# Autodesk Inventor assembly: Assemblage_chassis_14_11_C
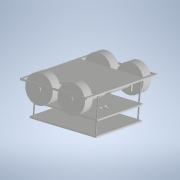
[picture p0: Inventor's stored thumbnail of the model, 180x180]
Saved by Autodesk Inventor 2020.1 (Build 241239000, 239)
## iProperties
Created: 2019-11-14
Part Number: Assemblage_chassis_14_11_C
Document SubType Name: Assembly
Designer: Admin
Author: Admin
## Documents named in this file (7)
- C:\Users\Admin\Desktop\Projet OrangeLab\CAO\Assemblage_chassis_14_11_C.iam
- C:\Users\Admin\Desktop\Projet OrangeLab\CAO\Chassis.ipt
- C:\Users\Admin\Desktop\Projet OrangeLab\CAO\Entretoises 80mm.ipt
- C:\Users\Admin\Desktop\Projet OrangeLab\CAO\Etage 1.ipt
- C:\Users\Admin\Desktop\Projet OrangeLab\CAO\Etage 2.ipt
- C:\Users\Admin\Desktop\Projet OrangeLab\CAO\Entretoises 50mm.ipt
- C:\Users\Admin\Desktop\Projet OrangeLab\CAO\Roue_moteur_C.iam
## Components (15 placed, 6 different names)
1. Chassis:1 — Mate:9, Mate:10, Mate:11, Mate:12, Mate:13, Mate:14, Mate:15, Mate:16, Mate:31, Mate:32, Mate:33, Mate:34, Mate:35, Mate:36, Mate:37, Mate:38, Mate:39, Mate:40, Mate:41, Mate:42
2. Entretoises 80mm:1 — Mate:12, Mate:13
3. Entretoises 80mm:2 — Mate:9, Mate:14, Mate:18
4. Entretoises 80mm:3 — Mate:11, Mate:15, Mate:17, Mate:19
5. Entretoises 80mm:4 — Mate:10, Mate:16
6. Etage 1:1 — Mate:17, Mate:18, Mate:19, Mate:20, Mate:21, Mate:22, Mate:23, Mate:24, Mate:25, Mate:26, Mate:27
7. Etage 2:1 — Mate:28, Mate:29, Mate:30
8. Entretoises 50mm:1 — Mate:20, Mate:21
9. Entretoises 50mm:2 — Mate:24, Mate:25, Mate:29, Mate:30
10. Entretoises 50mm:3 — Mate:26, Mate:27
11. Entretoises 50mm:4 — Mate:22, Mate:23, Mate:28
12. Roue_moteur_C:1 [sub-assembly] — Mate:31, Mate:32, Mate:33
13. Roue_moteur_C:2 [sub-assembly] — Mate:34, Mate:35, Mate:36
14. Roue_moteur_C:3 [sub-assembly] — Mate:40, Mate:41, Mate:42
15. Roue_moteur_C:4 [sub-assembly] — Mate:37, Mate:38, Mate:39
## Relationships (34: Mate 34)
- Mate:9: Chassis:1 ↔ Entretoises 80mm:2
- Mate:10: Chassis:1 ↔ Entretoises 80mm:4
- Mate:11: Chassis:1 ↔ Entretoises 80mm:3
- Mate:12: Chassis:1 ↔ Entretoises 80mm:1
- Mate:13: Chassis:1 ↔ Entretoises 80mm:1
- Mate:14: Chassis:1 ↔ Entretoises 80mm:2
- Mate:15: Chassis:1 ↔ Entretoises 80mm:3
- Mate:16: Chassis:1 ↔ Entretoises 80mm:4
- Mate:17: Entretoises 80mm:3 ↔ Etage 1:1
- Mate:18: Entretoises 80mm:2 ↔ Etage 1:1
- Mate:19: Entretoises 80mm:3 ↔ Etage 1:1
- Mate:20: Etage 1:1 ↔ Entretoises 50mm:1
- Mate:21: Etage 1:1 ↔ Entretoises 50mm:1
- Mate:22: Etage 1:1 ↔ Entretoises 50mm:4
- Mate:23: Etage 1:1 ↔ Entretoises 50mm:4
- Mate:24: Etage 1:1 ↔ Entretoises 50mm:2
- Mate:25: Etage 1:1 ↔ Entretoises 50mm:2
- Mate:26: Etage 1:1 ↔ Entretoises 50mm:3
- Mate:27: Etage 1:1 ↔ Entretoises 50mm:3
- Mate:28: Etage 2:1 ↔ Entretoises 50mm:4
- Mate:29: Etage 2:1 ↔ Entretoises 50mm:2
- Mate:30: Etage 2:1 ↔ Entretoises 50mm:2
- Mate:31: Chassis:1 ↔ Roue_moteur_C:1
- Mate:32: Chassis:1 ↔ Roue_moteur_C:1
- Mate:33: Chassis:1 ↔ Roue_moteur_C:1
- Mate:34: Chassis:1 ↔ Roue_moteur_C:2
- Mate:35: Chassis:1 ↔ Roue_moteur_C:2
- Mate:36: Chassis:1 ↔ Roue_moteur_C:2
- Mate:37: Chassis:1 ↔ Roue_moteur_C:4
- Mate:38: Chassis:1 ↔ Roue_moteur_C:4
- Mate:39: Chassis:1 ↔ Roue_moteur_C:4
- Mate:40: Chassis:1 ↔ Roue_moteur_C:3
- Mate:41: Chassis:1 ↔ Roue_moteur_C:3
- Mate:42: Chassis:1 ↔ Roue_moteur_C:3
